# Autodesk Inventor assembly: MiddleOfGripperWithPlate
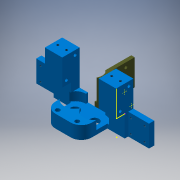
[picture p0: Inventor's stored thumbnail of the model, 180x180]
Saved by Autodesk Inventor 2019 (Build 230136000, 136)
## iProperties
Created: 2019-10-11
Part Number: MiddleOfGripperWithPlate
Document SubType Name: Assembly
Designer: james
Author: james
## Documents named in this file (3)
- F:\JimsDesign\Jims2020FTC\MiddleOfGripperWithPlate.iam
- F:\JimsDesign\Jims2020FTC\MiddleOfGripper.ipt
- F:\JimsDesign\Jims2020FTC\GripperSidePlateCarved.ipt
## Components (2 placed, 2 different names)
1. MiddleOfGripper:1 — Mate:2, Mate:3, Mate:4
2. GripperSidePlateCarved:1 — Mate:2, Mate:3, Mate:4
## Relationships (3: Mate 3)
- Mate:2: MiddleOfGripper:1 ↔ GripperSidePlateCarved:1
- Mate:3: MiddleOfGripper:1 ↔ GripperSidePlateCarved:1
- Mate:4: MiddleOfGripper:1 ↔ GripperSidePlateCarved:1
